# Autodesk Inventor assembly: robot scrivi
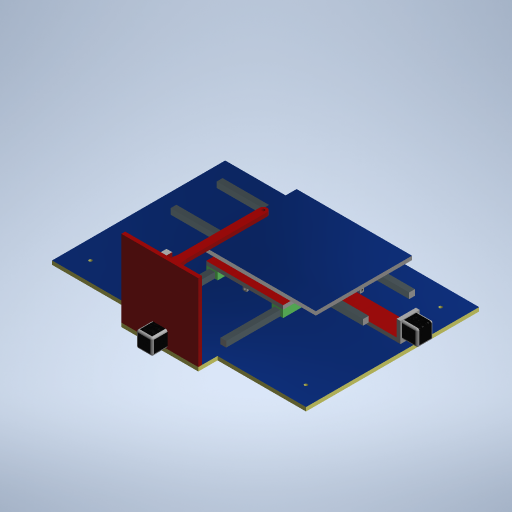
[picture p0: Inventor's stored thumbnail of the model, 512x512]
Saved by Autodesk Inventor 2024 (Build 280153000, 153)
## iProperties
Created: 2023-12-23
Part Number: robot scrivi
Document SubType Name: Assembly
Designer: Giorgio
Mass: 4367.81 g
Surface Area: 9701.46 cm^2
Volume: 4367.81 cm^3
Density: 1 g/cm^3
Author: Giorgio
## Documents named in this file (13)
- C:\Users\Giorgio\OneDrive\Desktop\me\inventor\robot scrivi.iam
- C:\Users\Giorgio\OneDrive\Desktop\me\inventor\base di lavoro.ipt
- C:\Users\Giorgio\OneDrive\Desktop\me\inventor\cuscinetto.ipt
- C:\Users\Public\Documents\Autodesk\Inventor 2024\guida.ipt
- C:\Users\Giorgio\OneDrive\Desktop\me\inventor\base sotto.ipt
- C:\Users\Giorgio\OneDrive\Desktop\me\inventor\guide corte y.ipt
- C:\Users\Giorgio\OneDrive\Desktop\me\inventor\base .ipt
- C:\Users\Giorgio\OneDrive\Desktop\me\inventor\piano z.ipt
- C:\Users\Giorgio\OneDrive\Desktop\me\inventor\guida z.ipt
- C:\Users\Giorgio\OneDrive\Desktop\me\inventor\porta penna.ipt
- C:\Users\Giorgio\OneDrive\Desktop\me\inventor\porta vite senza fine.ipt
- C:\Users\Giorgio\OneDrive\Desktop\me\inventor\staffa motore.ipt
- C:\Users\Giorgio\OneDrive\Desktop\me\inventor\motoreù.ipt
## Components (24 placed, 12 different names)
1. base di lavoro:1 — Coincidente:1, Coincidente:2, Coincidente:3, Coincidente:4, Allineato:5, Allineato:6, Allineato:7, Allineato:8, Allineato:34, Coincidente:26
2. cuscinetto:1 — Coincidente:1, Allineato:2, Allineato:3, Coincidente:7
3. cuscinetto:2 — Coincidente:3, Allineato:1, Allineato:4, Allineato:7
4. cuscinetto:3 — Coincidente:4, Allineato:2, Allineato:4, Allineato:5, Allineato:6
5. cuscinetto:4 — Coincidente:2, Allineato:1, Allineato:3, Allineato:8, Coincidente:5, Coincidente:6
6. guida:1 — Coincidente:5, Coincidente:6, Allineato:9, Allineato:10, Coincidente:8, Allineato:11
7. guida:2 — Allineato:9, Allineato:10, Coincidente:7, Allineato:12
8. base sotto:1 — Coincidente:8, Allineato:11, Allineato:12, Coincidente:9, Coincidente:10, Coincidente:11, Coincidente:12, Allineato:13, Allineato:16, Allineato:17, Allineato:18, Coincidente:28, Allineato:37, Allineato:39, Coincidente:29, Allineato:40, Allineato:41, Allineato:46
9. cuscinetto:5 — Coincidente:10, Allineato:13, Allineato:14, Allineato:15, Allineato:16, Coincidente:13
10. cuscinetto:6 — Coincidente:9, Allineato:14, Allineato:18, Allineato:19
11. cuscinetto:7 — Coincidente:11, Allineato:15, Allineato:17, Allineato:20, Coincidente:14
12. cuscinetto:8 — Coincidente:12, Allineato:19, Allineato:20, Coincidente:15, Coincidente:16
13. guide corte y:1 — Allineato:21, Allineato:22, Coincidente:13, Coincidente:14
14. guide corte y:2 — Allineato:21, Allineato:22, Coincidente:15, Coincidente:16, Coincidente:17, Allineato:23, Allineato:24
15. base :1 — Coincidente:17, Allineato:23, Allineato:24, Allineato:28, Coincidente:18, Coincidente:19, Allineato:42
16. piano z:1 — Allineato:28, Coincidente:18, Coincidente:19, Coincidente:20, Allineato:29, Allineato:30, Coincidente:31, Allineato:43
17. guida z:1 — Coincidente:20, Allineato:29, Allineato:30, Coincidente:21, Coincidente:22
18. cuscinetto:9 — Coincidente:21, Coincidente:22, Coincidente:23, Coincidente:24, Allineato:31
19. porta penna:1 — Coincidente:23, Coincidente:24, Allineato:31
20. porta vite senza fine:2 — Coincidente:28, Allineato:37, Allineato:39
21. porta vite senza fine:5 — Allineato:34, Coincidente:26
22. staffa motore:1 — Coincidente:29, Allineato:40, Allineato:41, Coincidente:30, Allineato:45
23. motoreù:1 — Coincidente:30, Allineato:45, Allineato:46
24. motoreù:2 — Coincidente:31, Allineato:42, Allineato:43
## Relationships (66: Flush 37, Mate 29)
- Coincidente:1 [Mate] (-1 mm): base di lavoro:1 ↔ cuscinetto:1
- Coincidente:2 [Mate]: base di lavoro:1 ↔ cuscinetto:4
- Coincidente:3 [Mate]: base di lavoro:1 ↔ cuscinetto:2
- Coincidente:4 [Mate]: base di lavoro:1 ↔ cuscinetto:3
- Allineato:1 [Flush]: cuscinetto:2 ↔ cuscinetto:4
- Allineato:2 [Flush]: cuscinetto:1 ↔ cuscinetto:3
- Allineato:3 [Flush]: cuscinetto:1 ↔ cuscinetto:4
- Allineato:4 [Flush]: cuscinetto:2 ↔ cuscinetto:3
- Allineato:5 [Flush] (-50 mm): base di lavoro:1 ↔ cuscinetto:3
- Allineato:6 [Flush] (50 mm): base di lavoro:1 ↔ cuscinetto:3
- Allineato:7 [Flush] (50 mm): base di lavoro:1 ↔ cuscinetto:2
- Allineato:8 [Flush] (-50 mm): base di lavoro:1 ↔ cuscinetto:4
- Coincidente:5 [Mate]: cuscinetto:4 ↔ guida:1
- Coincidente:6 [Mate]: cuscinetto:4 ↔ guida:1
- Allineato:9 [Flush]: guida:1 ↔ guida:2
- Allineato:10 [Flush]: guida:1 ↔ guida:2
- Coincidente:7 [Mate]: cuscinetto:1 ↔ guida:2
- Coincidente:8 [Mate]: guida:1 ↔ base sotto:1
- Allineato:11 [Flush] (150 mm): guida:1 ↔ base sotto:1
- Allineato:12 [Flush] (-7.5 mm): guida:2 ↔ base sotto:1
- Coincidente:9 [Mate]: base sotto:1 ↔ cuscinetto:6
- Coincidente:10 [Mate]: base sotto:1 ↔ cuscinetto:5
- Coincidente:11 [Mate]: base sotto:1 ↔ cuscinetto:7
- Coincidente:12 [Mate]: base sotto:1 ↔ cuscinetto:8
- Allineato:13 [Flush]: base sotto:1 ↔ cuscinetto:5
- Allineato:14 [Flush]: cuscinetto:5 ↔ cuscinetto:6
- Allineato:15 [Flush]: cuscinetto:5 ↔ cuscinetto:7
- Allineato:16 [Flush]: base sotto:1 ↔ cuscinetto:5
- Allineato:17 [Flush]: base sotto:1 ↔ cuscinetto:7
- Allineato:18 [Flush]: base sotto:1 ↔ cuscinetto:6
- Allineato:19 [Flush]: cuscinetto:6 ↔ cuscinetto:8
- Allineato:20 [Flush]: cuscinetto:7 ↔ cuscinetto:8
- Allineato:21 [Flush]: guide corte y:1 ↔ guide corte y:2
- Allineato:22 [Flush]: guide corte y:1 ↔ guide corte y:2
- Coincidente:13 [Mate]: cuscinetto:5 ↔ guide corte y:1
- Coincidente:14 [Mate]: cuscinetto:7 ↔ guide corte y:1
- Coincidente:15 [Mate]: cuscinetto:8 ↔ guide corte y:2
- Coincidente:16 [Mate]: cuscinetto:8 ↔ guide corte y:2
- Coincidente:17 [Mate]: guide corte y:2 ↔ base :1
- Allineato:23 [Flush] (237.5 mm): guide corte y:2 ↔ base :1
- Allineato:24 [Flush] (-30 mm): guide corte y:2 ↔ base :1
- Allineato:28 [Flush]: base :1 ↔ piano z:1
- Coincidente:18 [Mate] (-200 mm): base :1 ↔ piano z:1
- Coincidente:19 [Mate]: base :1 ↔ piano z:1
- Coincidente:20 [Mate]: piano z:1 ↔ guida z:1
- Allineato:29 [Flush]: piano z:1 ↔ guida z:1
- Allineato:30 [Flush] (92.55 mm): piano z:1 ↔ guida z:1
- Coincidente:21 [Mate]: guida z:1 ↔ cuscinetto:9
- Coincidente:22 [Mate]: guida z:1 ↔ cuscinetto:9
- Coincidente:23 [Mate]: cuscinetto:9 ↔ porta penna:1
- Coincidente:24 [Mate]: cuscinetto:9 ↔ porta penna:1
- Allineato:31 [Flush]: cuscinetto:9 ↔ porta penna:1
- Allineato:34 [Flush]: base di lavoro:1 ↔ porta vite senza fine:5
- Coincidente:26 [Mate]: base di lavoro:1 ↔ porta vite senza fine:5
- Coincidente:28 [Mate]: base sotto:1 ↔ porta vite senza fine:2
- Allineato:37 [Flush]: base sotto:1 ↔ porta vite senza fine:2
- Allineato:39 [Flush] (95 mm): base sotto:1 ↔ porta vite senza fine:2
- Coincidente:29 [Mate]: base sotto:1 ↔ staffa motore:1
- Allineato:40 [Flush]: base sotto:1 ↔ staffa motore:1
- Allineato:41 [Flush]: base sotto:1 ↔ staffa motore:1
- Coincidente:30 [Mate]: staffa motore:1 ↔ motoreù:1
- Coincidente:31 [Mate]: piano z:1 ↔ motoreù:2
- Allineato:42 [Flush] (12 mm): base :1 ↔ motoreù:2
- Allineato:43 [Flush] (80 mm): piano z:1 ↔ motoreù:2
- Allineato:45 [Flush] (2 mm): staffa motore:1 ↔ motoreù:1
- Allineato:46 [Flush] (4 mm): base sotto:1 ↔ motoreù:1
## Named parameters: Finish10_Area = 123.083, Finish10_Thickness = 0.05 mm, Finish11_Area = 112.593, Finish11_Thickness = 0.05 mm, Finish1_Area = 1264.62, Finish1_Thickness = 0.05 mm, Finish2_Area = 1264.62, Finish2_Thickness = 0.05 mm, Finish3_Area = 149.8, Finish3_Thickness = 0.05 mm, Finish4_Area = 449.4, Finish4_Thickness = 0.05 mm, Finish5_Area = 348.66, Finish5_Thickness = 0.05 mm, Finish6_Area = 6134.46, Finish6_Thickness = 0.05 mm, Finish7_Area = 3817.23, Finish7_Thickness = 0.05 mm, Finish8_Area = 163.721, Finish8_Thickness = 0.05 mm, Finish9_Area = 896.328, Finish9_Thickness = 0.05 mm
note: some values were not read from the file. Shown as the stored number, unit unknown: "Finish10_Area", "Finish11_Area", "Finish1_Area", "Finish2_Area", "Finish3_Area", "Finish4_Area", "Finish5_Area", "Finish6_Area", "Finish7_Area", "Finish8_Area", "Finish9_Area".
